# Autodesk Inventor assembly: Сборка под облегченный вариант
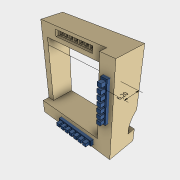
[picture p0: Inventor's stored thumbnail of the model, 180x180]
Saved by Autodesk Inventor 2021.2 (Build 252289000, 289)
## iProperties
Created: 2025-10-29
Part Number: Сборка под облегченный вариант
Document SubType Name: Assembly
Designer: Захаров
Author: Захаров
## Documents named in this file (3)
- C:\Users\User\Documents\CaseARHead1\Сборка под облегченный вариант.iam
- C:\Users\User\Documents\CaseARHead1\ЛЦМК.00002.00.00.00.00.01.ipt
- C:\Users\User\Documents\CaseARHead1\ЛЦМК000002.00.00.00.00.06-07.ipt
## Components (3 placed, 2 different names)
1. ЛЦМК000002.00.00.00.00.06-07:1 — Заподлицо:1, Совмещение:1, Заподлицо:2, Заподлицо:3, Заподлицо:4, Совмещение:2
2. ЛЦМК.00002.00.00.00.00.01:1 — Заподлицо:1, Совмещение:1, Заподлицо:2
3. ЛЦМК.00002.00.00.00.00.01:2 — Заподлицо:3, Заподлицо:4, Совмещение:2
## Relationships (6: Flush 4, Mate 2)
- Заподлицо:1 [Flush] (-3.2 mm): ЛЦМК000002.00.00.00.00.06-07:1 ↔ ЛЦМК.00002.00.00.00.00.01:1
- Совмещение:1 [Mate] (1 mm): ЛЦМК000002.00.00.00.00.06-07:1 ↔ ЛЦМК.00002.00.00.00.00.01:1
- Заподлицо:2 [Flush] (1.8 mm): ЛЦМК000002.00.00.00.00.06-07:1 ↔ ЛЦМК.00002.00.00.00.00.01:1
- Заподлицо:3 [Flush] (-6.2 mm): ЛЦМК000002.00.00.00.00.06-07:1 ↔ ЛЦМК.00002.00.00.00.00.01:2
- Заподлицо:4 [Flush] (1.8 mm): ЛЦМК000002.00.00.00.00.06-07:1 ↔ ЛЦМК.00002.00.00.00.00.01:2
- Совмещение:2 [Mate] (2 mm): ЛЦМК000002.00.00.00.00.06-07:1 ↔ ЛЦМК.00002.00.00.00.00.01:2
